# Autodesk Inventor assembly: ENSAMBLE COMPLETO PRUEBA
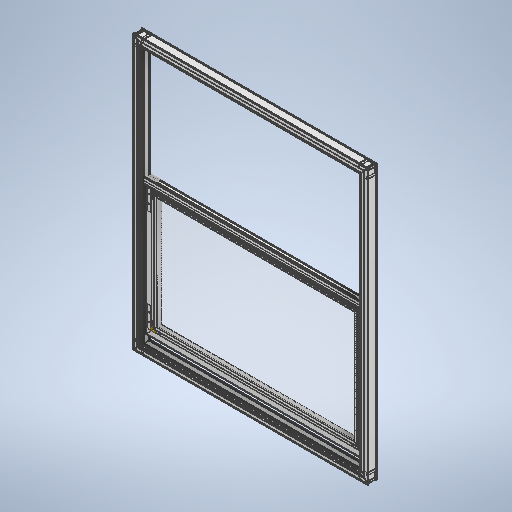
[picture p0: Inventor's stored thumbnail of the model, 512x512]
Saved by Autodesk Inventor 2025 (Build 290162000, 162)
## iProperties
Created: 2026-02-26
Part Number: ENSAMBLE COMPLETO PRUEBA
Document SubType Name: Assembly
Designer: Frank
Author: Frank
## Documents named in this file (4)
- C:\Users\Frank\OneDrive\CARPINTERIA ALUMINIO\PUERTAS Y VENTANAS\VENTANAS\ENSAMBLE COMPLETO PRUEBA.iam
- C:\Users\Frank\OneDrive\CARPINTERIA ALUMINIO\PUERTAS Y VENTANAS\VENTANAS\MARCOS\ENSAMBLES\MARCO CORREDERA SP40-09 EXT 1400x1200.iam
- MARCO CORREDERA SP40-09 EXT 1400x1200.iam
- C:\Users\Frank\OneDrive\CARPINTERIA ALUMINIO\PUERTAS Y VENTANAS\VENTANAS\VENTANAS\ENSAMBLES\HOJA CORREDERA SP40-10 EXT 1400x1200 - IZQUIERDA DELANTERA.iam
## Components (2 placed, 2 different names)
1. MARCO CORREDERA SP40-09 EXT 1400x1200:1 [sub-assembly] — Coincidencia:1, Nivelación:1, Nivelación:2, Nivelación:3, Nivelación:4
2. HOJA CORREDERA SP40-10 EXT 1400x1200 - IZQUIERDA DELANTERA:1 [sub-assembly] — Nivelación:3, Nivelación:4
## Relationships (5: Flush 4, Mate 1)
- Coincidencia:1 [Mate]: MARCO CORREDERA SP40-09 EXT 1400x1200:1
- Nivelación:1 [Flush]: MARCO CORREDERA SP40-09 EXT 1400x1200:1
- Nivelación:2 [Flush]: MARCO CORREDERA SP40-09 EXT 1400x1200:1
- Nivelación:3 [Flush]: MARCO CORREDERA SP40-09 EXT 1400x1200:1 ↔ HOJA CORREDERA SP40-10 EXT 1400x1200 - IZQUIERDA DELANTERA:1
- Nivelación:4 [Flush]: MARCO CORREDERA SP40-09 EXT 1400x1200:1 ↔ HOJA CORREDERA SP40-10 EXT 1400x1200 - IZQUIERDA DELANTERA:1
